# Autodesk Inventor assembly: manta ray assembly
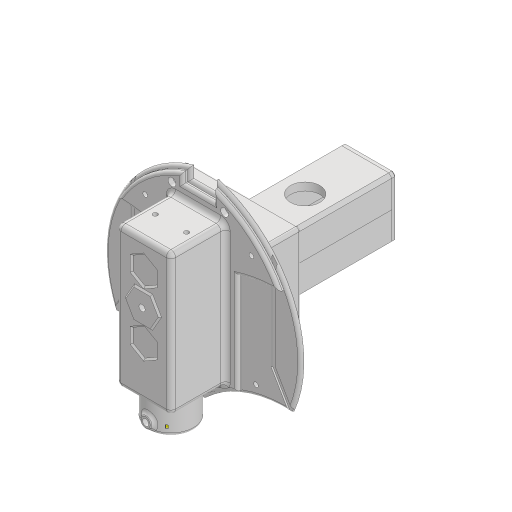
[picture p0: Inventor's stored thumbnail of the model, 512x512]
Saved by Autodesk Inventor 2024 (Build 280153000, 153)
## iProperties
Created: 2024-01-12
Part Number: manta ray assembly
Document SubType Name: Assembly
Designer: chris
Author: chris
## Documents named in this file (8)
- C:\Users\chris\Desktop\VTECH Semester 12\Hobby\Manta Ray\manta ray assembly.iam
- C:\Users\chris\Desktop\VTECH Semester 12\Hobby\Manta Ray\manta ray baseplate.ipt
- C:\Users\chris\Desktop\VTECH Semester 12\Hobby\Manta Ray\manta ray battery pack.ipt
- C:\Users\chris\Desktop\VTECH Semester 12\Hobby\Manta Ray\manta ray top plate.ipt
- C:\Users\chris\Desktop\VTECH Semester 12\Hobby\Manta Ray\manta ray_handle2.ipt
- C:\Users\chris\Desktop\VTECH Semester 12\Hobby\Manta Ray\manta ray_handle1.ipt
- C:\Users\chris\Desktop\VTECH Semester 12\Hobby\Manta Ray\manta ray handle cap.ipt
- C:\Users\chris\Desktop\VTECH Semester 12\Hobby\Manta Ray\manta ray cap.ipt
## Components (7 placed, 7 different names)
1. manta ray baseplate:1 — Rotational:1, Rotational:2, Rotational:3, Rotational:4
2. manta ray battery pack:1 — Rotational:1, Rotational:2, Rotational:5, Rotational:6, Rotational:7, Rotational:8
3. manta ray top plate:1 — Rotational:3, Rotational:4, Rotational:11
4. manta ray_handle2:1 — Rotational:7, Rotational:8, Rotational:9
5. manta ray_handle1:1 — Rotational:5, Rotational:6, Rotational:10
6. manta ray handle cap:1 — Rotational:9, Rotational:10
7. manta ray cap:1 — Rotational:11
## Relationships (11: RevoluteJoint 11)
- Rotational:1 [RevoluteJoint]: manta ray baseplate:1 ↔ manta ray battery pack:1
- Rotational:2 [RevoluteJoint]: manta ray baseplate:1 ↔ manta ray battery pack:1
- Rotational:3 [RevoluteJoint]: manta ray baseplate:1 ↔ manta ray top plate:1
- Rotational:4 [RevoluteJoint]: manta ray baseplate:1 ↔ manta ray top plate:1
- Rotational:5 [RevoluteJoint]: manta ray battery pack:1 ↔ manta ray_handle1:1
- Rotational:6 [RevoluteJoint]: manta ray battery pack:1 ↔ manta ray_handle1:1
- Rotational:7 [RevoluteJoint]: manta ray battery pack:1 ↔ manta ray_handle2:1
- Rotational:8 [RevoluteJoint]: manta ray battery pack:1 ↔ manta ray_handle2:1
- Rotational:9 [RevoluteJoint]: manta ray_handle2:1 ↔ manta ray handle cap:1
- Rotational:10 [RevoluteJoint]: manta ray_handle1:1 ↔ manta ray handle cap:1
- Rotational:11 [RevoluteJoint]: manta ray top plate:1 ↔ manta ray cap:1
